# Autodesk Inventor assembly: Outer_Tube_Adjst_Asm
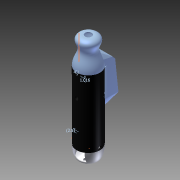
[picture p0: Inventor's stored thumbnail of the model, 180x180]
Saved by Autodesk Inventor 2011 SP2 (Build 150309200, 309)
## iProperties
Created: 2012-06-08
Part Number: Outer_Tube_Adjst_Asm
Document SubType Name: Assembly
Designer: sungwook
Author: sungwook
## Documents named in this file (4)
- C:\Users\sungwook\Documents\Inventor\Micron20_Base_Tube_Adjst\Outer_Tube_Adjst_Asm.iam
- C:\Users\sungwook\Documents\Inventor\Micron20_Base_Tube_Adjst\Outer_Tube.ipt
- C:\Users\sungwook\Documents\Inventor\Micron20_Base_Tube_Adjst\Parts\Handle\Ver2(Al_RP)\Handle_2_Back_rev2.ipt
- C:\Users\sungwook\Documents\Inventor\Micron20_Base_Tube_Adjst\Parts\Handle\Ver2(Al_RP)\Handle_2_Rev_Front.ipt
## Components (3 placed, 3 different names)
1. Outer_Tube:1 — Mate:1, Mate:2, Mate:3, Mate:4, Mate:5
2. Handle_2_Back_rev2:1 — Mate:1, Mate:2, Mate:5, Flush:6
3. Handle_2_Rev_Front:1 — Mate:3, Flush:4, Mate:4, Flush:6
## Relationships (7: Mate 5, Flush 2)
- Mate:1: Outer_Tube:1 ↔ Handle_2_Back_rev2:1
- Mate:2: Outer_Tube:1 ↔ Handle_2_Back_rev2:1
- Mate:3: Outer_Tube:1 ↔ Handle_2_Rev_Front:1
- Flush:4: Handle_2_Rev_Front:1
- Mate:4: Outer_Tube:1 ↔ Handle_2_Rev_Front:1
- Mate:5: Outer_Tube:1 ↔ Handle_2_Back_rev2:1
- Flush:6: Handle_2_Back_rev2:1 ↔ Handle_2_Rev_Front:1
